# Autodesk Inventor assembly: assembly
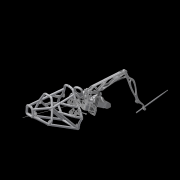
[picture p0: Inventor's stored thumbnail of the model, 180x180]
Saved by Autodesk Inventor 2020 (Build 240168000, 168)
## iProperties
Created: 2020-03-24
Part Number: assembly
Document SubType Name: Assembly
Designer: valer
Author: valer
## Documents named in this file (22)
- C:\Users\valer\Desktop\drummingrobot\src\Robot.iam
- C:\Users\valer\Desktop\drummingrobot\src\Chest.ipt
- C:\Users\valer\Desktop\drummingrobot\src\HeadScaled.ipt
- C:\Users\valer\Desktop\drummingrobot\src\UpperArm.ipt
- C:\Users\valer\Desktop\drummingrobot\src\UpperArmBracket.ipt
- C:\Users\valer\Desktop\drummingrobot\src\external\ShoulderConnectingRod.ipt
- C:\Users\valer\Desktop\drummingrobot\src\Forearm.ipt
- C:\Users\valer\Desktop\drummingrobot\src\external\Drumstick.ipt
- C:\Users\valer\Desktop\drummingrobot\src\external\ForearmShaftCollar.ipt
- C:\Users\valer\Desktop\drummingrobot\src\external\RodEndFixed.ipt
- C:\Users\valer\Desktop\drummingrobot\src\ShoulderBracket.ipt
- C:\Users\valer\Desktop\drummingrobot\src\ChestShoulderBracket.ipt
- C:\Users\valer\Desktop\drummingrobot\src\ChestShoulderBracketMirror.ipt
- C:\Users\valer\Desktop\drummingrobot\src\external\UpperArmActuatorBody.ipt
- C:\Users\valer\Desktop\drummingrobot\src\external\UpperArmActuatorShaft.ipt
- C:\Users\valer\Desktop\drummingrobot\src\external\ForearmActuatorBody.ipt
- C:\Users\valer\Desktop\drummingrobot\src\external\ForearmActuatorShaft.ipt
- C:\Users\valer\Desktop\drummingrobot\src\external\Drums.ipt
- C:\Users\valer\Desktop\drummingrobot\src\ForearmActuatorConnector.ipt
- C:\Users\valer\Desktop\drummingrobot\src\external\ArmRotationServoBody.ipt
- C:\Users\valer\Desktop\drummingrobot\src\external\ArmRotationServoHead.ipt
- C:\Users\valer\Desktop\drummingrobot\src\UpperArmActuatorBracket.ipt
## Components (47 placed, 21 different names)
1. Chest:1 — Angle:6, Mate:117, Mate:118, Mate:119, Mate:120, Mate:121, Mate:122, Mate:130, Mate:131, Mate:132, Mate:133, Mate:134, Mate:157, Angle:12
2. HeadScaled:1 — Angle:6
3. ChestConnectingRod:1 — Mate:88, Mate:89, Mate:105
4. ChestConnectingRod:2 — Mate:86, Mate:87, Mate:104
5. ChestConnectingRod:3 — Mate:84, Mate:85, Mate:98
6. ChestConnectingRod:4 — Mate:82, Mate:83, Mate:97
7. Drumstick:1 — Mate:79, Flush:3
8. ShaftCollar1/2:1 — Mate:79, Flush:3, Mate:236, Flush:18
9. RodEnd1/4-1/4-1:1 — Mate:82, Mate:281
10. RodEnd1/4-1/4-1:2 — Mate:83, Mate:97, Mate:123, Mate:125
11. RodEnd1/4-1/4-1:3 — Mate:84, Mate:280
12. RodEnd1/4-1/4-1:4 — Mate:85, Mate:98, Mate:124, Mate:142
13. RodEnd1/4-1/4-1:5 — Mate:86, Mate:283
14. RodEnd1/4-1/4-1:6 — Mate:87, Mate:104, Mate:126, Mate:129
15. RodEnd1/4-1/4-1:7 — Mate:88, Mate:284
16. RodEnd1/4-1/4-1:8 — Mate:89, Mate:105, Mate:127, Mate:128
17. ShoulderBracket:3 — Flush:22, Mate:280, Mate:281, Mate:285
18. ChestShoulderBracket:1 — Mate:120, Mate:121, Mate:122, Mate:123, Mate:124, Mate:125, Mate:142, Flush:22
19. ChestShoulderBracketMirror:1 — Mate:117, Mate:118, Mate:119, Mate:126, Mate:127, Mate:128, Mate:129
20. ChestShoulderBracket:2 — Mate:130, Mate:131, Mate:157, Mate:160, Mate:162, Mate:213, Mate:214
21. ChestShoulderBracketMirror:2 — Mate:132, Mate:133, Mate:134, Mate:141, Mate:146, Mate:148, Mate:149
22. ChestConnectingRod:5
23. ChestConnectingRod:6
24. RodEnd1/4-1/4-1:9
25. RodEnd1/4-1/4-1:10 — Mate:148, Mate:149
26. RodEnd1/4-1/4-1:11
27. RodEnd1/4-1/4-1:12 — Mate:141, Mate:146
28. ChestConnectingRod:7
29. ChestConnectingRod:8
30. RodEnd1/4-1/4-1:13
31. RodEnd1/4-1/4-1:14 — Mate:162, Mate:214
32. RodEnd1/4-1/4-1:15
33. RodEnd1/4-1/4-1:16 — Mate:160, Mate:213
34. UpperArmActuatorBody:1 — Mate:182, Mate:183, Mate:276
35. Forearm:1 — Flush:17, Mate:227, Mate:236, Flush:18, Mate:239, Mate:244
36. UpperArmActuatorShaft:2 — Mate:182, Mate:183, Mate:238, Flush:20
37. ForearmActuatorBody:1 — Mate:231, Mate:232, Mate:234, Flush:19
38. Drums:1 — Flush:13
39. ForearmActuatorShaft:3 — Flush:17, Mate:231, Mate:232, Mate:241, Mate:243, Angle:10, Mate:246
40. UpperArm:3 — Mate:227, Mate:234, Mate:238, Flush:19, Flush:20, Mate:249, Mate:250
41. ForearmActuatorConnector:1 — Mate:239, Mate:241, Mate:245, Angle:10, Mate:246
42. ForearmActuatorConnector:2 — Mate:243, Mate:244, Mate:245
43. UpperArmBracket:5 — Mate:249, Mate:250, Mate:272, Mate:274, Mate:275
44. ArmRotationServoBody:1 — Mate:258, Mate:259, Angle:12, Mate:285, Mate:286
45. ArmRotationServoHead:1 — Mate:258, Mate:259, Mate:273, Mate:277
46. UpperArmActuatorBracket:1 — Mate:272, Mate:273, Mate:274, Mate:275, Mate:276, Mate:277
47. ShoulderBracket:5 — Mate:283, Mate:284, Mate:286
## Relationships (93: Mate 83, Flush 7, Angle 3)
- Angle:6 (0 deg): Chest:1 ↔ HeadScaled:1
- Mate:79: Drumstick:1 ↔ ShaftCollar1/2:1
- Flush:3 (304.8 mm): Drumstick:1 ↔ ShaftCollar1/2:1
- Mate:82: ChestConnectingRod:4 ↔ RodEnd1/4-1/4-1:1
- Mate:83: ChestConnectingRod:4 ↔ RodEnd1/4-1/4-1:2
- Mate:84: ChestConnectingRod:3 ↔ RodEnd1/4-1/4-1:3
- Mate:85: ChestConnectingRod:3 ↔ RodEnd1/4-1/4-1:4
- Mate:86: ChestConnectingRod:2 ↔ RodEnd1/4-1/4-1:5
- Mate:87: ChestConnectingRod:2 ↔ RodEnd1/4-1/4-1:6
- Mate:88: ChestConnectingRod:1 ↔ RodEnd1/4-1/4-1:7
- Mate:89: ChestConnectingRod:1 ↔ RodEnd1/4-1/4-1:8
- Mate:97 (-25.4 mm): ChestConnectingRod:4 ↔ RodEnd1/4-1/4-1:2
- Mate:98 (-25.4 mm): ChestConnectingRod:3 ↔ RodEnd1/4-1/4-1:4
- Mate:104 (-25.4 mm): ChestConnectingRod:2 ↔ RodEnd1/4-1/4-1:6
- Mate:105 (-25.4 mm): ChestConnectingRod:1 ↔ RodEnd1/4-1/4-1:8
- Mate:117: Chest:1 ↔ ChestShoulderBracketMirror:1
- Mate:118: Chest:1 ↔ ChestShoulderBracketMirror:1
- Mate:119: Chest:1 ↔ ChestShoulderBracketMirror:1
- Mate:120: Chest:1 ↔ ChestShoulderBracket:1
- Mate:121: Chest:1 ↔ ChestShoulderBracket:1
- Mate:122: Chest:1 ↔ ChestShoulderBracket:1
- Mate:123: RodEnd1/4-1/4-1:2 ↔ ChestShoulderBracket:1
- Mate:124: RodEnd1/4-1/4-1:4 ↔ ChestShoulderBracket:1
- Mate:125: RodEnd1/4-1/4-1:2 ↔ ChestShoulderBracket:1
- Mate:126: RodEnd1/4-1/4-1:6 ↔ ChestShoulderBracketMirror:1
- Mate:127: RodEnd1/4-1/4-1:8 ↔ ChestShoulderBracketMirror:1
- Mate:128: RodEnd1/4-1/4-1:8 ↔ ChestShoulderBracketMirror:1
- Mate:129: RodEnd1/4-1/4-1:6 ↔ ChestShoulderBracketMirror:1
- Mate:130: Chest:1 ↔ ChestShoulderBracket:2
- Mate:131: Chest:1 ↔ ChestShoulderBracket:2
- Mate:132: Chest:1 ↔ ChestShoulderBracketMirror:2
- Mate:133: Chest:1 ↔ ChestShoulderBracketMirror:2
- Mate:134: Chest:1 ↔ ChestShoulderBracketMirror:2
- [Mate]: ChestConnectingRod:6 ↔ RodEnd1/4-1/4-1:9
- [Mate]: ChestConnectingRod:6 ↔ RodEnd1/4-1/4-1:10
- [Mate]: ChestConnectingRod:5 ↔ RodEnd1/4-1/4-1:11
- [Mate]: ChestConnectingRod:5 ↔ RodEnd1/4-1/4-1:12
- [Mate] (-25.4 mm): ChestConnectingRod:6 ↔ RodEnd1/4-1/4-1:10
- [Mate] (-25.4 mm): ChestConnectingRod:5 ↔ RodEnd1/4-1/4-1:12
- Mate:141: ChestShoulderBracketMirror:2 ↔ RodEnd1/4-1/4-1:12
- Mate:142: RodEnd1/4-1/4-1:4 ↔ ChestShoulderBracket:1
- Mate:146: ChestShoulderBracketMirror:2 ↔ RodEnd1/4-1/4-1:12
- Mate:148: ChestShoulderBracketMirror:2 ↔ RodEnd1/4-1/4-1:10
- Mate:149: ChestShoulderBracketMirror:2 ↔ RodEnd1/4-1/4-1:10
- [Mate]: ChestConnectingRod:8 ↔ RodEnd1/4-1/4-1:13
- [Mate]: ChestConnectingRod:8 ↔ RodEnd1/4-1/4-1:14
- [Mate]: ChestConnectingRod:7 ↔ RodEnd1/4-1/4-1:15
- [Mate]: ChestConnectingRod:7 ↔ RodEnd1/4-1/4-1:16
- [Mate] (-25.4 mm): ChestConnectingRod:8 ↔ RodEnd1/4-1/4-1:14
- [Mate] (-25.4 mm): ChestConnectingRod:7 ↔ RodEnd1/4-1/4-1:16
- Mate:157: Chest:1 ↔ ChestShoulderBracket:2
- Mate:160: ChestShoulderBracket:2 ↔ RodEnd1/4-1/4-1:16
- Mate:162: ChestShoulderBracket:2 ↔ RodEnd1/4-1/4-1:14
- Mate:182: UpperArmActuatorBody:1 ↔ UpperArmActuatorShaft:2
- Mate:183: UpperArmActuatorBody:1 ↔ UpperArmActuatorShaft:2
- Flush:13 (508 mm): Drums:1
- Mate:213: ChestShoulderBracket:2 ↔ RodEnd1/4-1/4-1:16
- Mate:214: ChestShoulderBracket:2 ↔ RodEnd1/4-1/4-1:14
- Flush:17: Forearm:1 ↔ ForearmActuatorShaft:3
- Mate:227: Forearm:1 ↔ UpperArm:3
- Mate:231: ForearmActuatorBody:1 ↔ ForearmActuatorShaft:3
- Mate:232: ForearmActuatorBody:1 ↔ ForearmActuatorShaft:3
- Mate:234: ForearmActuatorBody:1 ↔ UpperArm:3
- Mate:236: ShaftCollar1/2:1 ↔ Forearm:1
- Flush:18 (12.7 mm): ShaftCollar1/2:1 ↔ Forearm:1
- Mate:238: UpperArmActuatorShaft:2 ↔ UpperArm:3
- Flush:19: ForearmActuatorBody:1 ↔ UpperArm:3
- Flush:20: UpperArmActuatorShaft:2 ↔ UpperArm:3
- Mate:239: Forearm:1 ↔ ForearmActuatorConnector:1
- Mate:241: ForearmActuatorShaft:3 ↔ ForearmActuatorConnector:1
- Mate:243: ForearmActuatorShaft:3 ↔ ForearmActuatorConnector:2
- Mate:244: Forearm:1 ↔ ForearmActuatorConnector:2
- Mate:245: ForearmActuatorConnector:1 ↔ ForearmActuatorConnector:2
- Angle:10 (-180 deg): ForearmActuatorShaft:3 ↔ ForearmActuatorConnector:1
- Mate:246: ForearmActuatorShaft:3 ↔ ForearmActuatorConnector:1
- Mate:249: UpperArm:3 ↔ UpperArmBracket:5
- Mate:250: UpperArm:3 ↔ UpperArmBracket:5
- Mate:258: ArmRotationServoBody:1 ↔ ArmRotationServoHead:1
- Mate:259: ArmRotationServoBody:1 ↔ ArmRotationServoHead:1
- Angle:12 (0 deg): Chest:1 ↔ ArmRotationServoBody:1
- Mate:272: UpperArmBracket:5 ↔ UpperArmActuatorBracket:1
- Mate:273: ArmRotationServoHead:1 ↔ UpperArmActuatorBracket:1
- Mate:274: UpperArmBracket:5 ↔ UpperArmActuatorBracket:1
- Mate:275: UpperArmBracket:5 ↔ UpperArmActuatorBracket:1
- Mate:276: UpperArmActuatorBody:1 ↔ UpperArmActuatorBracket:1
- Mate:277: ArmRotationServoHead:1 ↔ UpperArmActuatorBracket:1
- Flush:22: ShoulderBracket:3 ↔ ChestShoulderBracket:1
- Mate:280: RodEnd1/4-1/4-1:3 ↔ ShoulderBracket:3
- Mate:281: RodEnd1/4-1/4-1:1 ↔ ShoulderBracket:3
- Mate:283: RodEnd1/4-1/4-1:5 ↔ ShoulderBracket:5
- Mate:284: RodEnd1/4-1/4-1:7 ↔ ShoulderBracket:5
- Mate:285: ShoulderBracket:3 ↔ ArmRotationServoBody:1
- Mate:286: ArmRotationServoBody:1 ↔ ShoulderBracket:5
## Named parameters: d244_d149 = 0 mm, d245_d150 = 0 mm, d246_d151 = 0 mm, d247_d152 = 0 mm, d248_d197 = -25.4 mm, d249_d198 = -25.4 mm, d259_d145 = 0 mm, d260_d146 = 0 mm, d261_d147 = 0 mm, d262_d148 = 0 mm, d263_d190 = -25.4 mm, d264_d191 = -25.4 mm
